# Autodesk Inventor assembly: elbowassembly
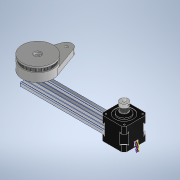
[picture p0: Inventor's stored thumbnail of the model, 180x180]
Saved by Autodesk Inventor 2022 (Build 260153000, 153)
## iProperties
Created: 2022-02-22
Part Number: elbowassembly
Document SubType Name: Assembly
Designer: JK
Author: JK
## Documents named in this file (7)
- C:\Users\JK\Documents\Inventor\ScaraNema\elbowassembly.iam
- C:\Users\JK\Documents\Inventor\ScaraNema\MOTOR_LONG.ipt
- C:\Users\JK\Documents\Inventor\ScaraNema\Inverse timing belt reducer\RoboDigg GT2 16 pulley.ipt
- C:\Users\JK\Documents\Inventor\ScaraNema\V-Slot 20x20\V-Slot 20x20x150.ipt
- C:\Users\JK\Documents\Inventor\ScaraNema\V-Slot 20x20.ipt
- C:\Users\JK\Documents\Inventor\ScaraNema\elbowpulley2.ipt
- C:\Users\JK\Documents\Inventor\ScaraNema\elbowsupport.ipt
## Components (5 placed, 5 different names)
1. MOTOR_LONG:1 — Coincidencia:1, Coincidencia:2, Nivelación:1, Nivelación:2, Coincidencia:3
2. RoboDigg GT2 16 pulley:1 — Coincidencia:1, Coincidencia:3, Nivelación:3
3. V-Slot 20x20x150:1 — Coincidencia:2, Nivelación:1, Nivelación:2
4. elbowpulley2:1 — Nivelación:3, Coincidencia:4
5. elbowsupport:1 — Coincidencia:4
## Relationships (7: Mate 4, Flush 3)
- Coincidencia:1 [Mate]: MOTOR_LONG:1 ↔ RoboDigg GT2 16 pulley:1
- Coincidencia:2 [Mate]: MOTOR_LONG:1 ↔ V-Slot 20x20x150:1
- Nivelación:1 [Flush] (10.75 mm): MOTOR_LONG:1 ↔ V-Slot 20x20x150:1
- Nivelación:2 [Flush]: MOTOR_LONG:1 ↔ V-Slot 20x20x150:1
- Coincidencia:3 [Mate] (3 mm): MOTOR_LONG:1 ↔ RoboDigg GT2 16 pulley:1
- Nivelación:3 [Flush]: RoboDigg GT2 16 pulley:1 ↔ elbowpulley2:1
- Coincidencia:4 [Mate]: elbowpulley2:1 ↔ elbowsupport:1
